# Autodesk Inventor assembly: Сборка1
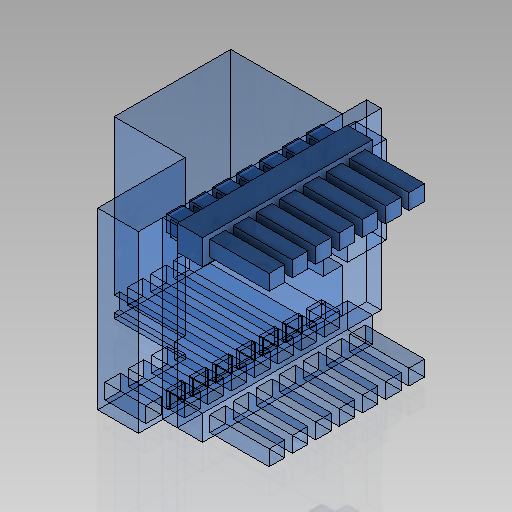
[picture p0: Inventor's stored thumbnail of the model, 512x512]
Saved by Autodesk Inventor 2021.2 (Build 252289000, 289)
## iProperties
Created: 2025-10-22
Part Number: Сборка1
Document SubType Name: Assembly
Designer: Захаров
Author: Захаров
## Documents named in this file (3)
- C:\Users\Public\Documents\Kingroon\Models\CaseARHead1\Сборка1.iam
- C:\Users\Public\Documents\Kingroon\Models\CaseARHead1\ЛЦМК.00002.00.00.00.00.01.ipt
- C:\Users\Public\Documents\Kingroon\Models\CaseARHead1\Сборка2.iam
## Components (3 placed, 2 different names)
1. ЛЦМК.00002.00.00.00.00.01:1
2. Сборка2:1 [sub-assembly] — Совмещение:1, Совмещение:2
3. ЛЦМК.00002.00.00.00.00.01:2 — Совмещение:1, Совмещение:2
## Relationships (2: Mate 2)
- Совмещение:1 [Mate]: Сборка2:1 ↔ ЛЦМК.00002.00.00.00.00.01:2
- Совмещение:2 [Mate]: Сборка2:1 ↔ ЛЦМК.00002.00.00.00.00.01:2
